# Autodesk Inventor assembly: LaundryRobot_v01
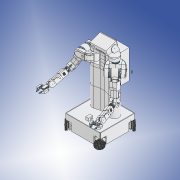
[picture p0: Inventor's stored thumbnail of the model, 180x180]
Saved by Autodesk Inventor 2017 SP1 (Build 210196100, 196)
## iProperties
Created: 2017-03-11
Part Number: LaundryRobot_v01
Document SubType Name: Assembly
Designer: zallen
Author: zallen
## Documents named in this file (4)
- C:\Users\Zach\Documents\GitHub\cr-laundry-robot\LaundryRobot_v01.iam
- C:\Users\Zach\Documents\GitHub\cr-laundry-robot\src\Body\Body.iam
- C:\Users\Zach\Documents\GitHub\cr-laundry-robot\src\Head\Head.iam
- C:\Users\Zach\Documents\GitHub\cr-laundry-robot\src\Base\Base.iam
## Components (3 placed, 3 different names)
1. Body:1 [sub-assembly] — Mate:7, Mate:18, Mate:20, Mate:21, Mate:22, Mate:24
2. Head:1 [sub-assembly] — Mate:7, Mate:18, Mate:20
3. Base:1 [sub-assembly] — Mate:11, Mate:12, Mate:21, Mate:22, Mate:23, Mate:24
## Relationships (9: Mate 9)
- Mate:7: Body:1 ↔ Head:1
- Mate:11: Base:1
- Mate:12: Base:1
- Mate:18: Body:1 ↔ Head:1
- Mate:20: Body:1 ↔ Head:1
- Mate:21: Body:1 ↔ Base:1
- Mate:22: Body:1 ↔ Base:1
- Mate:23: Base:1
- Mate:24: Body:1 ↔ Base:1
